# Autodesk Inventor assembly: robot
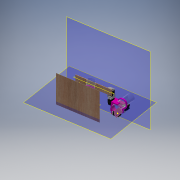
[picture p0: Inventor's stored thumbnail of the model, 180x180]
Saved by Autodesk Inventor 2017 (Build 210142000, 142)
## iProperties
Created: 2018-04-01
Part Number: robot
Document SubType Name: Assembly
Designer: franc
Mass: 1235.72 g
Surface Area: 6399.52 cm^2
Volume: 1204.8 cm^3
Density: 1.02566 g/cm^3
Author: franc
## Documents named in this file (7)
- C:\Users\franc\Desktop\EsialRobotik\Mecanique\2018\robot\robot.iam
- C:\Users\franc\Desktop\EsialRobotik\Mecanique\base_roulante\baseRoulante.iam
- C:\Users\franc\Desktop\EsialRobotik\Mecanique\2018\robot\socle-robot.ipt
- C:\Users\franc\Desktop\EsialRobotik\Mecanique\2018\robot\etage-bras.ipt
- C:\Users\franc\Desktop\EsialRobotik\Mecanique\2018\robot\traitement-eau\recuperation.iam
- C:\Users\franc\Desktop\EsialRobotik\Mecanique\2018\robot\traitement-eau\lanceur.iam
- C:\Users\franc\Desktop\EsialRobotik\Mecanique\2018\robot\equerre-bras.ipt
## Components (6 placed, 6 different names)
1. baseRoulante:1 [sub-assembly] — Affleurement:1, Affleurement:2, Placage:1, Angle:1, Placage:24, Affleurement:6
2. socle-robot:1 — Affleurement:1, Affleurement:2, Placage:1, Affleurement:3, Placage:22, Placage:27, Affleurement:5, Placage:28, Placage:32
3. etage-bras:1 — Affleurement:3, Angle:1, Placage:22, Placage:24, Placage:31, Placage:33, Affleurement:7, Affleurement:8
4. recuperation:1 [sub-assembly] — Placage:33, Affleurement:7, Affleurement:8
5. lanceur:1 [sub-assembly] — Placage:28, Placage:29, Placage:30, Placage:32
6. equerre-bras:1 — Placage:29, Placage:30, Placage:31
## Relationships (18: Mate 10, Flush 7, Angle 1)
- Affleurement:1 [Flush] (5 mm): baseRoulante:1 ↔ socle-robot:1
- Affleurement:2 [Flush] (54 mm): baseRoulante:1 ↔ socle-robot:1
- Placage:1 [Mate]: baseRoulante:1 ↔ socle-robot:1
- Affleurement:3 [Flush] (5 mm): socle-robot:1 ↔ etage-bras:1
- Angle:1 (0 deg): baseRoulante:1 ↔ etage-bras:1
- Placage:22 [Mate]: socle-robot:1 ↔ etage-bras:1
- Placage:24 [Mate] (172 mm): baseRoulante:1 ↔ etage-bras:1
- Placage:27 [Mate]: socle-robot:1
- Affleurement:5 [Flush]: socle-robot:1
- Placage:28 [Mate] (-150 mm): socle-robot:1 ↔ lanceur:1
- Placage:29 [Mate]: lanceur:1 ↔ equerre-bras:1
- Placage:30 [Mate]: lanceur:1 ↔ equerre-bras:1
- Placage:31 [Mate]: etage-bras:1 ↔ equerre-bras:1
- Placage:32 [Mate] (-100 mm): socle-robot:1 ↔ lanceur:1
- Affleurement:6 [Flush] (340 mm): baseRoulante:1
- Placage:33 [Mate]: etage-bras:1 ↔ recuperation:1
- Affleurement:7 [Flush]: etage-bras:1 ↔ recuperation:1
- Affleurement:8 [Flush]: etage-bras:1 ↔ recuperation:1
